# Autodesk Inventor assembly: AutinhhoAssembly
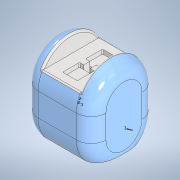
[picture p0: Inventor's stored thumbnail of the model, 180x180]
Saved by Autodesk Inventor 2020 (Build 240168000, 168)
## iProperties
Created: 2019-09-20
Part Number: AutinhhoAssembly
Document SubType Name: Assembly
Designer: Acer
Author: Acer
## Documents named in this file (3)
- C:\Users\Acer\Documents\Autinho\AutinhhoAssembly.iam
- C:\Users\Acer\Documents\Autinho\Autinho2.ipt
- C:\Users\Acer\Documents\Autinho\tela.iam
## Components (2 placed, 2 different names)
1. Autinho2:1 — Mate:1, Mate:3, Mate:4
2. tela:1 [sub-assembly] — Mate:1, Mate:3, Mate:4
## Relationships (3: Mate 3)
- Mate:1: Autinho2:1 ↔ tela:1
- Mate:3: Autinho2:1 ↔ tela:1
- Mate:4: Autinho2:1 ↔ tela:1
